# Autodesk Inventor assembly: RearLegsWithHip
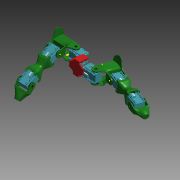
[picture p0: Inventor's stored thumbnail of the model, 180x180]
Saved by Autodesk Inventor 2015 (Build 190159000, 159)
## iProperties
Created: 2015-03-02
Part Number: RearLegsWithHip
Document SubType Name: Assembly
Designer: Henke
Author: Henke
## Documents named in this file (3)
- D:\Study_and_Projects\KTH\KEX i robotik\CAD\RearLegsWithHip.iam
- D:\Study_and_Projects\KTH\KEX i robotik\CAD\Leg3DOF.iam
- D:\Study_and_Projects\KTH\KEX i robotik\CAD\ButtConnector.ipt
## Components (3 placed, 2 different names)
1. Leg3DOF:1 [sub-assembly] — Mate:1
2. ButtConnector:1 — Mate:1, Mate:4, Flush:2
3. Leg3DOF:2 [sub-assembly] — Mate:4
## Relationships (3: Mate 2, Flush 1)
- Mate:1: Leg3DOF:1 ↔ ButtConnector:1
- Mate:4: ButtConnector:1 ↔ Leg3DOF:2
- Flush:2: ButtConnector:1
